# Autodesk Inventor assembly: 바퀴풀리결합_8PI
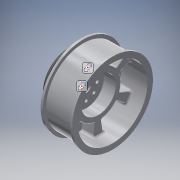
[picture p0: Inventor's stored thumbnail of the model, 180x180]
Saved by Autodesk Inventor 2017 (Build 210142000, 142)
## iProperties
Part Number: 바퀴풀리결합_8PI
Material: 일반
Document SubType Name: Assembly
Designer: minom
Author: minom
## Documents named in this file (3)
- C:\Users\minom\Documents\Inventor\Projects\2017 IRC Sumo Mino ver.2\바퀴풀리결합_8PI.iam
- C:\Users\minom\Documents\Inventor\Projects\2017 IRC Sumo Mino ver.2\바퀴8PI.ipt
- C:\Users\minom\Documents\Inventor\Projects\2017 IRC Sumo Mino ver.2\ATP25XL025-A-N8-KC90-QFC20-M3-FC45_0-TPC3_b.ipt
## Components (2 placed, 2 different names)
1. 바퀴8PI:1 — 메이트:2, 메이트:3, 메이트:4
2. ATP25XL025-A-N8-KC90-QFC20-M3-FC45_0-TPC3_b:1 — 메이트:2, 메이트:3, 메이트:4
## Relationships (3: Mate 3)
- 메이트:2 [Mate]: 바퀴8PI:1 ↔ ATP25XL025-A-N8-KC90-QFC20-M3-FC45_0-TPC3_b:1
- 메이트:3 [Mate]: 바퀴8PI:1 ↔ ATP25XL025-A-N8-KC90-QFC20-M3-FC45_0-TPC3_b:1
- 메이트:4 [Mate]: 바퀴8PI:1 ↔ ATP25XL025-A-N8-KC90-QFC20-M3-FC45_0-TPC3_b:1
